# Autodesk Inventor assembly: case
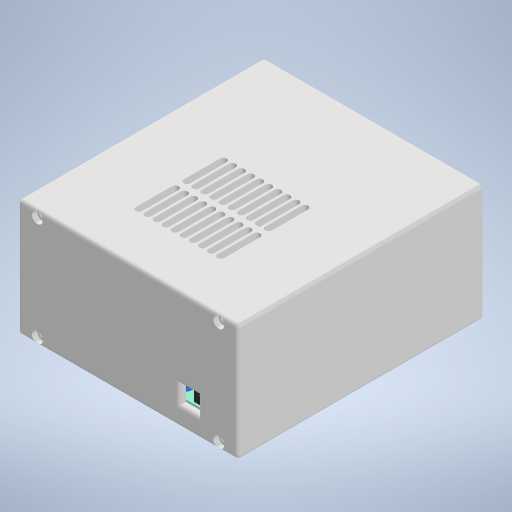
[picture p0: Inventor's stored thumbnail of the model, 512x512]
Saved by Autodesk Inventor 2023 (Build 270158000, 158)
## iProperties
Created: 2022-12-05
Part Number: case
Document SubType Name: Assembly
Designer: elect
Author: elect
## Documents named in this file (7)
- C:\Users\elect\JDC\Electronics\Projects\Mil_Time_Clock\model\FreeCAD\CASE_ASSM\case.iam
- C:\Users\elect\JDC\Electronics\Projects\Mil_Time_Clock\model\FreeCAD\MCU_IPT\MCU_pcb-MCU_BOARD.iam
- C:\Users\elect\JDC\Electronics\Projects\Mil_Time_Clock\model\FreeCAD\DISPLAY_IPT\DISPLAY_pcb-LED_DISPLAY_BOARD.iam
- C:\Users\elect\JDC\Electronics\Projects\Mil_Time_Clock\model\FreeCAD\Case_Front.ipt
- C:\Users\elect\JDC\Electronics\Projects\Mil_Time_Clock\model\FreeCAD\Case_lens.ipt
- C:\Users\elect\JDC\Electronics\Projects\Mil_Time_Clock\model\FreeCAD\Case_Rear.ipt
- C:\Users\elect\JDC\Electronics\Projects\Mil_Time_Clock\model\FreeCAD\button.ipt
## Components (10 placed, 6 different names)
1. MCU_pcb-MCU_BOARD:1 [sub-assembly] — Mate:1, Mate:2, Flush:1
2. DISPLAY_pcb-LED_DISPLAY_BOARD:1 [sub-assembly] — Mate:1, Mate:2, Flush:1, Mate:6, Mate:7
3. Case_Front:1 — Mate:3, Mate:4, Mate:5, Mate:6, Mate:7, Mate:8, Flush:2, Flush:3, Mate:9, Mate:10, Mate:11, Mate:12, Mate:13, Mate:14, Mate:15, Mate:16, Mate:17, Mate:18
4. Case_lens:1 — Mate:3, Mate:4, Mate:5
5. Case_Rear:1 — Mate:8, Flush:2, Flush:3
6. button:1 — Mate:9, Mate:18
7. button:2 — Mate:11, Mate:17
8. button:3 — Mate:10, Mate:14
9. button:4 — Mate:13, Mate:16
10. button:5 — Mate:12, Mate:15
## Relationships (21: Mate 18, Flush 3)
- Mate:1 (1.27 mm): MCU_pcb-MCU_BOARD:1 ↔ DISPLAY_pcb-LED_DISPLAY_BOARD:1
- Mate:2: MCU_pcb-MCU_BOARD:1 ↔ DISPLAY_pcb-LED_DISPLAY_BOARD:1
- Flush:1 (-8.9154 mm): MCU_pcb-MCU_BOARD:1 ↔ DISPLAY_pcb-LED_DISPLAY_BOARD:1
- Mate:3: Case_Front:1 ↔ Case_lens:1
- Mate:4: Case_Front:1 ↔ Case_lens:1
- Mate:5: Case_Front:1 ↔ Case_lens:1
- Mate:6: DISPLAY_pcb-LED_DISPLAY_BOARD:1 ↔ Case_Front:1
- Mate:7: DISPLAY_pcb-LED_DISPLAY_BOARD:1 ↔ Case_Front:1
- Mate:8: Case_Front:1 ↔ Case_Rear:1
- Flush:2: Case_Front:1 ↔ Case_Rear:1
- Flush:3: Case_Front:1 ↔ Case_Rear:1
- Mate:9: Case_Front:1 ↔ button:1
- Mate:10: Case_Front:1 ↔ button:3
- Mate:11: Case_Front:1 ↔ button:2
- Mate:12: Case_Front:1 ↔ button:5
- Mate:13: Case_Front:1 ↔ button:4
- Mate:14: Case_Front:1 ↔ button:3
- Mate:15: Case_Front:1 ↔ button:5
- Mate:16: Case_Front:1 ↔ button:4
- Mate:17: Case_Front:1 ↔ button:2
- Mate:18: Case_Front:1 ↔ button:1
